# Autodesk Inventor assembly: ForeArm_without_hand
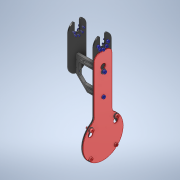
[picture p0: Inventor's stored thumbnail of the model, 180x180]
Saved by Autodesk Inventor 2022.3 (Build 263350000, 350)
## iProperties
Created: 2022-01-11
Part Number: ForeArm_without_hand
Document SubType Name: Assembly
Designer: Masato Kubotera
Author: Masato Kubotera
## Documents named in this file (9)
- C:\Users\Masato\Documents\Inventor\Inventor for CIT Brains\SUSTAINA-OP\UpperBody\Arm\ForeArm_without_hand.iam
- C:\Users\Masato\Documents\Inventor\Inventor for CIT Brains\SUSTAINA-OP\UpperBody\Arm\ForeArm_outside_frame.ipt
- C:\Users\Masato\Documents\Inventor\Inventor for CIT Brains\SUSTAINA-OP\UpperBody\Arm\ForeArm_inside_frame.ipt
- C:\Users\Masato\Documents\Inventor\Inventor for CIT Brains\SUSTAINA-OP\ReadyMade\Screw\UC-0306.ipt
- C:\Users\Masato\Documents\Inventor\Inventor for CIT Brains\SUSTAINA-OP\ReadyMade\Screw\UC-2606.ipt
- C:\Users\Masato\Documents\Inventor\Inventor for CIT Brains\SUSTAINA-OP\UpperBody\Arm\ForeArm_outside_cloth.ipt
- C:\Users\Masato\Documents\Inventor\Inventor for CIT Brains\SUSTAINA-OP\ReadyMade\Bush\L3040-8110TB.ipt
- C:\Users\Masato\Documents\Inventor\Inventor for CIT Brains\SUSTAINA-OP\ReadyMade\Screw\UC-0308.ipt
- C:\Users\Masato\Documents\Inventor\Inventor for CIT Brains\SUSTAINA-OP\UpperBody\Arm\ForeArm_diagonal.iam
## Components (25 placed, 8 different names)
1. ForeArm_inside_frame:1 — 挿入:29, 挿入:30, 挿入:35, 挿入:36, 挿入:37, 挿入:38, 挿入:40, Insert:52, Insert:53
2. ForeArm_outside_frame:1 — 挿入:16, 挿入:17, 挿入:28, 挿入:31, 挿入:32, 挿入:33, 挿入:34, メイト:1, メイト:2, フラッシュ:1, 挿入:39, 挿入:41, 挿入:42, 挿入:43, Insert:54
3. ForeArm_outside_cloth:1 — 挿入:47, 挿入:48, 挿入:49
4. L3040-8110TB:1 — 挿入:41, 挿入:47, 挿入:50
5. L3040-8110TB:2 — 挿入:42, 挿入:48, 挿入:51
6. L3040-8110TB:3 — 挿入:43, 挿入:46, 挿入:49
7. ForeArm_diagonal:1 [sub-assembly] — Insert:52, Insert:53, Insert:54
8. UC-2606:1 — 挿入:31
9. UC-2606:2 — 挿入:32
10. UC-2606:3 — 挿入:33
11. UC-2606:4 — 挿入:34
12. UC-2606:5 — 挿入:35
13. UC-2606:6 — 挿入:36
14. UC-2606:7 — 挿入:37
15. UC-2606:8 — 挿入:38
16. UC-2606:9 — 挿入:39
17. UC-2606:10 — 挿入:40
18. UC-0308:1 — 挿入:46
19. UC-0308:2 — 挿入:50
20. UC-0308:3 — 挿入:51
21. UC-0306:1 — 挿入:16
22. UC-0306:2 — 挿入:17
23. UC-0306:3 — 挿入:28
24. UC-0306:10 — 挿入:30
25. UC-0306:5 — 挿入:29
## Relationships (30: Insert 27, Mate 2, Flush 1)
- 挿入:16 [Insert]: ForeArm_outside_frame:1 ↔ UC-0306:1
- 挿入:17 [Insert]: ForeArm_outside_frame:1 ↔ UC-0306:2
- 挿入:28 [Insert]: ForeArm_outside_frame:1 ↔ UC-0306:3
- 挿入:29 [Insert]: ForeArm_inside_frame:1 ↔ UC-0306:5
- 挿入:30 [Insert]: ForeArm_inside_frame:1 ↔ UC-0306:10
- 挿入:31 [Insert]: ForeArm_outside_frame:1 ↔ UC-2606:1
- 挿入:32 [Insert]: ForeArm_outside_frame:1 ↔ UC-2606:2
- 挿入:33 [Insert]: ForeArm_outside_frame:1 ↔ UC-2606:3
- 挿入:34 [Insert]: ForeArm_outside_frame:1 ↔ UC-2606:4
- 挿入:35 [Insert]: ForeArm_inside_frame:1 ↔ UC-2606:5
- 挿入:36 [Insert]: ForeArm_inside_frame:1 ↔ UC-2606:6
- 挿入:37 [Insert]: ForeArm_inside_frame:1 ↔ UC-2606:7
- 挿入:38 [Insert]: ForeArm_inside_frame:1 ↔ UC-2606:8
- メイト:1 [Mate]: ForeArm_outside_frame:1
- メイト:2 [Mate]: ForeArm_outside_frame:1
- フラッシュ:1 [Flush]: ForeArm_outside_frame:1
- 挿入:39 [Insert]: ForeArm_outside_frame:1 ↔ UC-2606:9
- 挿入:40 [Insert]: ForeArm_inside_frame:1 ↔ UC-2606:10
- 挿入:41 [Insert]: ForeArm_outside_frame:1 ↔ L3040-8110TB:1
- 挿入:42 [Insert]: ForeArm_outside_frame:1 ↔ L3040-8110TB:2
- 挿入:43 [Insert]: ForeArm_outside_frame:1 ↔ L3040-8110TB:3
- 挿入:46 [Insert]: L3040-8110TB:3 ↔ UC-0308:1
- 挿入:47 [Insert]: ForeArm_outside_cloth:1 ↔ L3040-8110TB:1
- 挿入:48 [Insert]: ForeArm_outside_cloth:1 ↔ L3040-8110TB:2
- 挿入:49 [Insert]: ForeArm_outside_cloth:1 ↔ L3040-8110TB:3
- 挿入:50 [Insert]: L3040-8110TB:1 ↔ UC-0308:2
- 挿入:51 [Insert]: L3040-8110TB:2 ↔ UC-0308:3
- Insert:52: ForeArm_inside_frame:1 ↔ ForeArm_diagonal:1
- Insert:53: ForeArm_inside_frame:1 ↔ ForeArm_diagonal:1
- Insert:54: ForeArm_outside_frame:1 ↔ ForeArm_diagonal:1
